# Autodesk Inventor assembly: RaspberryCameraV2InCase
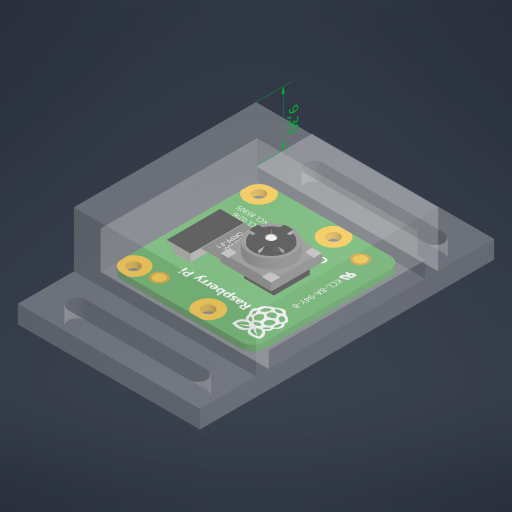
[picture p0: Inventor's stored thumbnail of the model, 512x512]
Saved by Autodesk Inventor 2023 (Build 270158030, 158C)
## iProperties
Created: 2022-07-13
Part Number: RaspberryCameraV2InCase
Document SubType Name: Assembly
Designer: Norbert Ligas
Author: Norbert Ligas
## Documents named in this file (3)
- C:\Users\norbe\Repozytoria\NormalMapScanner\3D_modeling\construction\parts\board_box\RaspberryCameraV2InCase.iam
- C:\Users\norbe\Repozytoria\NormalMapScanner\3D_modeling\construction\parts\board_box\RaspberryCameraV2Case.ipt
- C:\Users\norbe\Repozytoria\NormalMapScanner\3D_modeling\construction\parts\board_box\RaspberryPiCameraV2.ipt
## Components (2 placed, 2 different names)
1. RaspberryCameraV2Case:1 — Mate:1, Mate:2, Mate:3, Flush:2, Flush:3
2. RaspberryPiCameraV2:1 — Mate:1, Mate:4, Flush:1
## Relationships (7: Mate 4, Flush 3)
- Mate:1: RaspberryCameraV2Case:1 ↔ RaspberryPiCameraV2:1
- Mate:2: RaspberryCameraV2Case:1
- Mate:3: RaspberryCameraV2Case:1
- Mate:4: RaspberryPiCameraV2:1
- Flush:1: RaspberryPiCameraV2:1
- Flush:2: RaspberryCameraV2Case:1
- Flush:3: RaspberryCameraV2Case:1
